# Autodesk Inventor assembly: doveTailTestAssembly
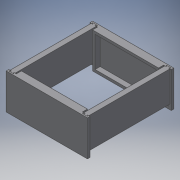
[picture p0: Inventor's stored thumbnail of the model, 180x180]
Saved by Autodesk Inventor 2016 (Build 200138000, 138)
## iProperties
Created: 2015-11-04
Part Number: doveTailTestAssembly
Document SubType Name: Assembly
Designer: rossmosier
Author: rossmosier
## Documents named in this file (4)
- C:\Users\rossmosier\Documents\CAD Team\CADTeam\Assemblies\doveTailTestAssembly.iam
- C:\Users\rossmosier\Documents\CAD Team\CADTeam\Parts\doveTailOtherSide.ipt
- C:\Users\rossmosier\Documents\CAD Team\CADTeam\Parts\doveTailSide.ipt
- C:\Users\rossmosier\Documents\CAD Team\CADTeam\Parts\doveTailBar.ipt
## Components (4 placed, 3 different names)
1. doveTailOtherSide:1 — Mate:2
2. doveTailSide:1 — Mate:1, Mate:3
3. doveTailBar:2 — Mate:1, Mate:2
4. doveTailBar:3 — Mate:3
## Relationships (3: Mate 3)
- Mate:1: doveTailSide:1 ↔ doveTailBar:2
- Mate:2: doveTailOtherSide:1 ↔ doveTailBar:2
- Mate:3: doveTailSide:1 ↔ doveTailBar:3
